# Autodesk Inventor assembly: Adrian_Drehteller
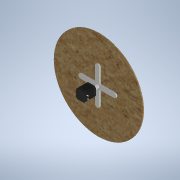
[picture p0: Inventor's stored thumbnail of the model, 180x180]
Saved by Autodesk Inventor 2021 (Build 250183000, 183)
## iProperties
Created: 2022-07-12
Part Number: Adrian_Drehteller
Document SubType Name: Assembly
Designer: adria
Mass: 596.176 g
Surface Area: 2962.29 cm^2
Volume: 746.973 cm^3
Density: 0.798123 g/cm^3
Author: adria
## Documents named in this file (4)
- C:\Users\adria\OneDrive - tum.de\G2_Waste-Recycling\CAD\Adrian_Drehteller.iam
- C:\Users\adria\OneDrive - tum.de\G2_Waste-Recycling\CAD\stepper-motor-nema17-simplified-model-1.snapshot.3\motor.ipt
- C:\Users\adria\OneDrive - tum.de\G2_Waste-Recycling\CAD\Adapter_drehteller.iam
- C:\Users\adria\OneDrive - tum.de\G2_Waste-Recycling\CAD\Drehteller.ipt
## Components (3 placed, 3 different names)
1. motor:1 — Passend:1, Passend:2, Winkel:1
2. Adapter_drehteller:1 [sub-assembly] — Passend:1, Passend:2, Winkel:1, Passend:3, Passend:4
3. Drehteller:1 — Passend:3, Passend:4
## Relationships (5: Mate 4, Angle 1)
- Passend:1 [Mate]: motor:1 ↔ Adapter_drehteller:1
- Passend:2 [Mate]: motor:1 ↔ Adapter_drehteller:1
- Winkel:1 [Angle] (0 deg): motor:1 ↔ Adapter_drehteller:1
- Passend:3 [Mate]: Adapter_drehteller:1 ↔ Drehteller:1
- Passend:4 [Mate]: Adapter_drehteller:1 ↔ Drehteller:1
